# Autodesk Inventor assembly: ship
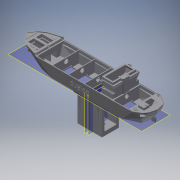
[picture p0: Inventor's stored thumbnail of the model, 180x180]
Saved by Autodesk Inventor 2018 (Build 220112000, 112)
## iProperties
Created: 2017-10-27
Part Number: ship
Document SubType Name: Assembly
Designer: erwin
Author: erwin
## Documents named in this file (3)
- D:\GitHub\SSJeVoisWheeledCargoShip\design\ship.iam
- D:\GitHub\SSJeVoisWheeledCargoShip\design\hull.ipt
- D:\GitHub\SSJeVoisWheeledCargoShip\design\holder.ipt
## Components (2 placed, 2 different names)
1. hull:1 — Flush:1, Flush:2
2. holder:1 — Flush:1, Flush:2
## Relationships (2: Flush 2)
- Flush:1: hull:1 ↔ holder:1
- Flush:2: hull:1 ↔ holder:1
